# Autodesk Inventor assembly: Cockpit_
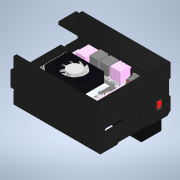
[picture p0: Inventor's stored thumbnail of the model, 180x180]
Saved by Autodesk Inventor 2020.4 (Build 244396000, 396)
## iProperties
Created: 2022-01-06
Part Number: Cockpit_
Document SubType Name: Assembly
Designer: Masato Kubotera
Mass: 586.569 g
Surface Area: 2053.33 cm^2
Volume: 316.504 cm^3
Density: 1.85327 g/cm^3
Author: Masato Kubotera
## Documents named in this file (11)
- C:\Users\Masato\Documents\Inventor\CIT Brains_Inventor\OpenPlatform_ver3_0\UpperBody\Cockpit\Cockpit_.iam
- C:\Users\Masato\Documents\Inventor\CIT Brains_Inventor\OpenPlatform_ver3_0\UpperBody\Cockpit\Cockpit_side_frame.ipt
- C:\Users\Masato\Documents\Inventor\CIT Brains_Inventor\OpenPlatform_ver3_0\UpperBody\Cockpit\Cockpit_front_frame.ipt
- C:\Users\Masato\Documents\Inventor\CIT Brains_Inventor\OpenPlatform_ver3_0\UpperBody\Cockpit\Cockpit_bottom_frame.ipt
- C:\Users\Masato\Documents\Inventor\CIT Brains_Inventor\OpenPlatform_ver3_0\UpperBody\Cockpit\Cockpit_middle_frame.ipt
- C:\Users\Masato\Documents\Inventor\CIT Brains_Inventor\OpenPlatform_ver3_0\Ready_Made\KCD11-A-101011BB.ipt
- C:\Users\Masato\Documents\Inventor\CIT Brains_Inventor\OpenPlatform_ver3_0\UpperBody\Cockpit\MainBoard.ipt
- C:\Users\Masato\Documents\Inventor\CIT Brains_Inventor\OpenPlatform_ver3_0\Ready_Made\Jetson_Xavier_NX_DevKit_without_Wi-FiAntennas\Jetson_Xavier_NX_DevKit.ipt
- C:\Users\Masato\Documents\Inventor\CIT Brains_Inventor\OpenPlatform_ver3_0\Ready_Made\HP-G830C2800S3.ipt
- C:\Users\Masato\Documents\Inventor\CIT Brains_Inventor\OpenPlatform_ver3_0\UpperBody\Cockpit\Cockpit_top_frame.ipt
- C:\Users\Masato\Documents\Inventor\CIT Brains_Inventor\OpenPlatform_ver3_0\UpperBody\Cockpit\Cockpit_back_frame.ipt
## Components (10 placed, 10 different names)
1. Cockpit_side_frame:1 — 挿入:1, 挿入:2, 挿入:3, 挿入:4, 挿入:5, 挿入:6, フラッシュ:1, メイト:1, フラッシュ:2, メイト:2, メイト:3, メイト:4, フラッシュ:3, 挿入:13, 挿入:14, 挿入:15, 挿入:16
2. Cockpit_front_frame:1 — 挿入:1, 挿入:2
3. Cockpit_bottom_frame:1 — 挿入:3, 挿入:4, 挿入:9, 挿入:10
4. Cockpit_middle_frame:1 — 挿入:5, 挿入:6, 挿入:11, 挿入:12
5. KCD11-A-101011BB:1 — メイト:2, メイト:3, メイト:4
6. MainBoard:1 — 挿入:9, 挿入:10
7. Jetson_Xavier_NX_DevKit:1 — 挿入:11, 挿入:12
8. HP-G830C2800S3:1 — フラッシュ:3
9. Cockpit_top_frame:1 — 挿入:13, 挿入:14
10. Cockpit_back_frame:1 — 挿入:15, 挿入:16
## Relationships (21: Insert 14, Mate 4, Flush 3)
- 挿入:1 [Insert]: Cockpit_side_frame:1 ↔ Cockpit_front_frame:1
- 挿入:2 [Insert]: Cockpit_side_frame:1 ↔ Cockpit_front_frame:1
- 挿入:3 [Insert]: Cockpit_side_frame:1 ↔ Cockpit_bottom_frame:1
- 挿入:4 [Insert]: Cockpit_side_frame:1 ↔ Cockpit_bottom_frame:1
- 挿入:5 [Insert]: Cockpit_side_frame:1 ↔ Cockpit_middle_frame:1
- 挿入:6 [Insert]: Cockpit_side_frame:1 ↔ Cockpit_middle_frame:1
- フラッシュ:1 [Flush]: Cockpit_side_frame:1
- メイト:1 [Mate]: Cockpit_side_frame:1
- フラッシュ:2 [Flush]: Cockpit_side_frame:1
- メイト:2 [Mate] (0.05 mm): Cockpit_side_frame:1 ↔ KCD11-A-101011BB:1
- メイト:3 [Mate] (0.05 mm): Cockpit_side_frame:1 ↔ KCD11-A-101011BB:1
- メイト:4 [Mate]: Cockpit_side_frame:1 ↔ KCD11-A-101011BB:1
- 挿入:9 [Insert] (5 mm): Cockpit_bottom_frame:1 ↔ MainBoard:1
- 挿入:10 [Insert] (5 mm): Cockpit_bottom_frame:1 ↔ MainBoard:1
- 挿入:11 [Insert]: Cockpit_middle_frame:1 ↔ Jetson_Xavier_NX_DevKit:1
- 挿入:12 [Insert]: Cockpit_middle_frame:1 ↔ Jetson_Xavier_NX_DevKit:1
- フラッシュ:3 [Flush] (-5 mm): Cockpit_side_frame:1 ↔ HP-G830C2800S3:1
- 挿入:13 [Insert]: Cockpit_side_frame:1 ↔ Cockpit_top_frame:1
- 挿入:14 [Insert]: Cockpit_side_frame:1 ↔ Cockpit_top_frame:1
- 挿入:15 [Insert]: Cockpit_side_frame:1 ↔ Cockpit_back_frame:1
- 挿入:16 [Insert]: Cockpit_side_frame:1 ↔ Cockpit_back_frame:1
